# Autodesk Inventor assembly: mini Cryostat FOOT3
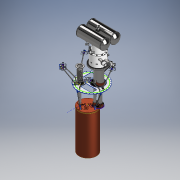
[picture p0: Inventor's stored thumbnail of the model, 180x180]
Saved by Autodesk Inventor 2018 (Build 220112000, 112)
## iProperties
Created: 2018-10-10
Part Number: mini Cryostat FOOT3
Document SubType Name: Assembly
Designer: Admin
Author: Admin
## Documents named in this file (12)
- C:\Users\freyja\Documents\Cryostat\CAD\mini Cryostat FOOT3.iam
- C:\Users\freyja\Documents\Cryostat\CAD\External Models\CH40415 24JUL14 C.ipt
- C:\Users\freyja\Documents\Cryostat\CAD\vacuum jacket long.ipt
- C:\Users\freyja\Documents\Cryostat\CAD\vacuum jacket.ipt
- C:\Users\freyja\Documents\Cryostat\CAD\Top Plate V2.2.ipt
- C:\Users\freyja\Documents\Cryostat\CAD\mini 55K stage.ipt
- C:\Users\freyja\Documents\Cryostat\CAD\foot type 3.iam
- C:\Users\freyja\Documents\Cryostat\CAD\Radiation Sheild 2K.ipt
- C:\Users\freyja\Documents\Cryostat\CAD\still pipe.iam
- C:\Users\freyja\Documents\Cryostat\CAD\4K shield2.iam
- C:\Users\freyja\Documents\Cryostat\CAD\2K8 FEET.iam
- C:\Users\freyja\Documents\Cryostat\CAD\2K8 FEET long.iam
## Components (20 placed, 11 different names)
1. Top Plate V2.2:1 — Mate:16, Mate:18, Mate:19, Mate:20, Mate:21, Mate:26, Mate:135, Mate:136, Mate:137, Mate:138, Mate:139, Mate:140, Mate:141, Mate:142, Mate:143, Mate:144, Mate:145, Mate:146, Mate:149, Mate:150, Mate:153, Mate:154, Mate:155, Mate:156
2. CH40415 24JUL14 C:1 — Mate:16, Mate:18, Mate:26, Mate:161, Mate:175
3. vacuum jacket long:1 — Mate:7, Mate:8, Mate:9
4. vacuum jacket:1 — Mate:7, Mate:8, Mate:9, Mate:19, Mate:20, Mate:21
5. mini 55K stage:1 — Mate:100, Mate:102, Mate:147, Mate:148, Mate:151, Mate:152, Mate:157, Mate:158, Mate:159, Mate:160, Mate:161, Mate:162, Mate:163, Mate:164, Mate:165, Mate:166, Mate:167, Mate:168, Mate:169, Mate:170, Mate:181, Mate:182, Mate:183, Mate:184, Mate:191, Mate:192, Mate:193, Mate:194
6. Radiation Sheild 2K:1 — Mate:100, Mate:102
7. still pipe:1 [sub-assembly] — Mate:135, Mate:136, Mate:162
8. foot type 3:1 [sub-assembly] — Mate:143, Mate:155, Mate:158, Mate:164
9. foot type 3:2 [sub-assembly] — Mate:140, Mate:153, Mate:159, Mate:169, Mate:173
10. foot type 3:3 [sub-assembly] — Mate:138, Mate:149, Mate:151, Mate:163
11. foot type 3:4 [sub-assembly] — Mate:144, Mate:154, Mate:160, Mate:168
12. foot type 3:5 [sub-assembly] — Mate:139, Mate:150, Mate:152, Mate:170
13. foot type 3:6 [sub-assembly] — Mate:137, Mate:145, Mate:148, Mate:166
14. foot type 3:7 [sub-assembly] — Mate:141, Mate:156, Mate:157, Mate:165, Mate:174
15. foot type 3:8 [sub-assembly] — Mate:142, Mate:146, Mate:147, Mate:167
16. 4K shield2:1 [sub-assembly] — Mate:175, Mate:177, Mate:178, Mate:185, Mate:186, Mate:187, Mate:188, Mate:189, Mate:190
17. 2K8 FEET:1 [sub-assembly] — Mate:177, Mate:181, Mate:183, Mate:186
18. 2K8 FEET:2 [sub-assembly] — Mate:178, Mate:182, Mate:184, Mate:185
19. 2K8 FEET long:1 [sub-assembly] — Mate:187, Mate:190, Mate:193, Mate:194
20. 2K8 FEET long:2 [sub-assembly] — Mate:188, Mate:189, Mate:191, Mate:192
## Relationships (66: Mate 66)
- Mate:7: vacuum jacket long:1 ↔ vacuum jacket:1
- Mate:8: vacuum jacket long:1 ↔ vacuum jacket:1
- Mate:9: vacuum jacket long:1 ↔ vacuum jacket:1
- Mate:16: Top Plate V2.2:1 ↔ CH40415 24JUL14 C:1
- Mate:18: Top Plate V2.2:1 ↔ CH40415 24JUL14 C:1
- Mate:19: Top Plate V2.2:1 ↔ vacuum jacket:1
- Mate:20: Top Plate V2.2:1 ↔ vacuum jacket:1
- Mate:21: Top Plate V2.2:1 ↔ vacuum jacket:1
- Mate:26: Top Plate V2.2:1 ↔ CH40415 24JUL14 C:1
- Mate:100: mini 55K stage:1 ↔ Radiation Sheild 2K:1
- Mate:102: mini 55K stage:1 ↔ Radiation Sheild 2K:1
- Mate:135: Top Plate V2.2:1 ↔ still pipe:1
- Mate:136: Top Plate V2.2:1 ↔ still pipe:1
- Mate:137: Top Plate V2.2:1 ↔ foot type 3:6
- Mate:138: Top Plate V2.2:1 ↔ foot type 3:3
- Mate:139: Top Plate V2.2:1 ↔ foot type 3:5
- Mate:140: Top Plate V2.2:1 ↔ foot type 3:2
- Mate:141: Top Plate V2.2:1 ↔ foot type 3:7
- Mate:142: Top Plate V2.2:1 ↔ foot type 3:8
- Mate:143: Top Plate V2.2:1 ↔ foot type 3:1
- Mate:144: Top Plate V2.2:1 ↔ foot type 3:4
- Mate:145: Top Plate V2.2:1 ↔ foot type 3:6
- Mate:146: Top Plate V2.2:1 ↔ foot type 3:8
- Mate:147: mini 55K stage:1 ↔ foot type 3:8
- Mate:148: mini 55K stage:1 ↔ foot type 3:6
- Mate:149: Top Plate V2.2:1 ↔ foot type 3:3
- Mate:150: Top Plate V2.2:1 ↔ foot type 3:5
- Mate:151: mini 55K stage:1 ↔ foot type 3:3
- Mate:152: mini 55K stage:1 ↔ foot type 3:5
- Mate:153: Top Plate V2.2:1 ↔ foot type 3:2
- Mate:154: Top Plate V2.2:1 ↔ foot type 3:4
- Mate:155: Top Plate V2.2:1 ↔ foot type 3:1
- Mate:156: Top Plate V2.2:1 ↔ foot type 3:7
- Mate:157: mini 55K stage:1 ↔ foot type 3:7
- Mate:158: mini 55K stage:1 ↔ foot type 3:1
- Mate:159: mini 55K stage:1 ↔ foot type 3:2
- Mate:160: mini 55K stage:1 ↔ foot type 3:4
- Mate:161: CH40415 24JUL14 C:1 ↔ mini 55K stage:1
- Mate:162: mini 55K stage:1 ↔ still pipe:1
- Mate:163: mini 55K stage:1 ↔ foot type 3:3
- Mate:164: mini 55K stage:1 ↔ foot type 3:1
- Mate:165: mini 55K stage:1 ↔ foot type 3:7
- Mate:166: mini 55K stage:1 ↔ foot type 3:6
- Mate:167: mini 55K stage:1 ↔ foot type 3:8
- Mate:168: mini 55K stage:1 ↔ foot type 3:4
- Mate:169: mini 55K stage:1 ↔ foot type 3:2
- Mate:170: mini 55K stage:1 ↔ foot type 3:5
- Mate:173: foot type 3:2
- Mate:174: foot type 3:7
- Mate:175 (3.81 mm): CH40415 24JUL14 C:1 ↔ 4K shield2:1
- Mate:177: 4K shield2:1 ↔ 2K8 FEET:1
- Mate:178: 4K shield2:1 ↔ 2K8 FEET:2
- Mate:181: mini 55K stage:1 ↔ 2K8 FEET:1
- Mate:182: mini 55K stage:1 ↔ 2K8 FEET:2
- Mate:183: mini 55K stage:1 ↔ 2K8 FEET:1
- Mate:184: mini 55K stage:1 ↔ 2K8 FEET:2
- Mate:185: 4K shield2:1 ↔ 2K8 FEET:2
- Mate:186: 4K shield2:1 ↔ 2K8 FEET:1
- Mate:187: 4K shield2:1 ↔ 2K8 FEET long:1
- Mate:188: 4K shield2:1 ↔ 2K8 FEET long:2
- Mate:189: 4K shield2:1 ↔ 2K8 FEET long:2
- Mate:190: 4K shield2:1 ↔ 2K8 FEET long:1
- Mate:191: mini 55K stage:1 ↔ 2K8 FEET long:2
- Mate:192: mini 55K stage:1 ↔ 2K8 FEET long:2
- Mate:193: mini 55K stage:1 ↔ 2K8 FEET long:1
- Mate:194: mini 55K stage:1 ↔ 2K8 FEET long:1
